# Autodesk Inventor assembly: манипулятогр
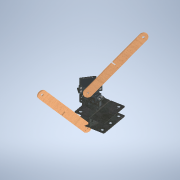
[picture p0: Inventor's stored thumbnail of the model, 180x180]
Saved by Autodesk Inventor 2020.1 (Build 241239000, 239)
## iProperties
Created: 2021-08-17
Part Number: манипулятогр
Document SubType Name: Assembly
Designer: Ni3na
Author: Ni3na
## Documents named in this file (4)
- C:\Users\Ni3na\Documents\GitHub\avatar-kvantoriada\3D\манипулятогр .iam
- C:\Users\Ni3na\Documents\GitHub\avatar-kvantoriada\3D\сборка серва.iam
- C:\Users\Ni3na\Documents\GitHub\avatar-kvantoriada\3D\Деталь1.ipt
- C:\Users\Ni3na\Documents\GitHub\avatar-kvantoriada\3D\основа.ipt
## Components (6 placed, 3 different names)
1. сборка серва:1 [sub-assembly] — Жесткий:1, Жесткий:3
2. сборка серва:2 [sub-assembly] — Жесткий:1, Жесткий:2
3. Деталь1:2 — Жесткий:2
4. Деталь1:3
5. основа:1 — Жесткий:3, Жесткий:4
6. основа:2 — Жесткий:4
## Relationships (4: WeldJoint 4)
- Жесткий:1 [WeldJoint]: сборка серва:1 ↔ сборка серва:2
- Жесткий:2 [WeldJoint]: сборка серва:2 ↔ Деталь1:2
- Жесткий:3 [WeldJoint]: сборка серва:1 ↔ основа:1
- Жесткий:4 [WeldJoint]: основа:1 ↔ основа:2
